# Autodesk Inventor assembly: Assembly - Before Cover
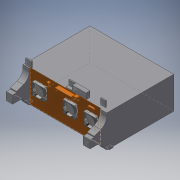
[picture p0: Inventor's stored thumbnail of the model, 180x180]
Saved by Autodesk Inventor 2017 (Build 210142000, 142)
## iProperties
Created: 2021-05-31
Part Number: Assembly - Before Cover
Document SubType Name: Assembly
Designer: Win240
Author: Win240
## Documents named in this file (4)
- C:\Users\Win240\Desktop\MASTER LiBCM Safety Cover\Assembly - Before Cover.iam
- C:\Users\Win240\Desktop\MASTER LiBCM Safety Cover\IMA Battery Case Primitive.ipt
- C:\Users\Win240\Desktop\MASTER LiBCM Safety Cover\PCB.ipt
- C:\Users\Win240\Desktop\MASTER LiBCM Safety Cover\Fan.ipt
## Components (5 placed, 3 different names)
1. IMA Battery Case Primitive:1 — Mate:1, Flush:1, Mate:2
2. PCB:1 — Mate:1, Flush:1, Mate:2, Insert:1, Insert:2, Insert:3, Insert:4, Insert:5, Insert:6
3. Fan:1 — Insert:1, Insert:6
4. Fan:2 — Insert:2, Insert:5
5. Fan:3 — Insert:3, Insert:4
## Relationships (9: Insert 6, Mate 2, Flush 1)
- Mate:1: IMA Battery Case Primitive:1 ↔ PCB:1
- Flush:1: IMA Battery Case Primitive:1 ↔ PCB:1
- Mate:2 (1.5 mm): IMA Battery Case Primitive:1 ↔ PCB:1
- Insert:1: PCB:1 ↔ Fan:1
- Insert:2: PCB:1 ↔ Fan:2
- Insert:3: PCB:1 ↔ Fan:3
- Insert:4: PCB:1 ↔ Fan:3
- Insert:5: PCB:1 ↔ Fan:2
- Insert:6: PCB:1 ↔ Fan:1
